# Autodesk Inventor assembly: Controller Asssembly
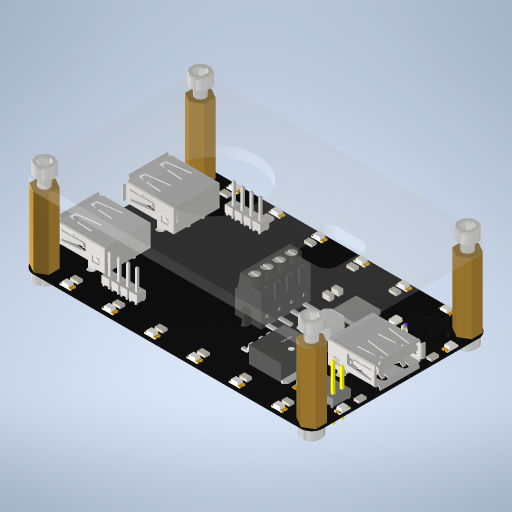
[picture p0: Inventor's stored thumbnail of the model, 512x512]
Saved by Autodesk Inventor 2023 (Build 270158000, 158)
## iProperties
Created: 2022-08-29
Part Number: Controller Asssembly
Document SubType Name: Assembly
Designer: swift
Author: swift
## Documents named in this file (5)
- C:\Users\swift\workspace\fairy-light-controller\Controller Cover\Controller Asssembly.iam
- C:\Users\swift\workspace\fairy-light-controller\Controller Cover\Fairy_Light_Controller_PCB_v1.ipt
- C:\Users\swift\workspace\fairy-light-controller\Controller Cover\Cover.ipt
- C:\Users\swift\workspace\fairy-light-controller\Controller Cover\Standoff.ipt
- C:\Users\swift\workspace\fairy-light-controller\Controller Cover\M3x6.ipt
## Components (14 placed, 4 different names)
1. Fairy_Light_Controller_PCB_v1:1 — Flush:1, Mate:1, Mate:2, Mate:3, Mate:4, Mate:5, Mate:6, Mate:16, Mate:17, Mate:18, Mate:19, Mate:20, Mate:21, Mate:22, Mate:23
2. Cover:1 — Mate:7, Mate:8, Mate:9, Mate:10, Mate:11, Mate:12, Mate:13, Mate:14, Mate:15
3. Standoff:1 — Flush:1, Flush:2, Mate:7
4. Standoff:2 — Mate:1, Mate:2, Flush:2, Angle:1
5. Standoff:3 — Mate:3, Mate:4, Flush:3
6. Standoff:4 — Mate:5, Mate:6, Flush:3
7. M3x6:1 — Mate:8, Mate:9, Flush:4, Angle:2, Flush:5
8. M3x6:2 — Mate:10, Mate:11, Angle:1, Flush:4, Angle:3, Flush:6
9. M3x6:3 — Mate:12, Mate:13, Angle:2, Flush:7
10. M3x6:4 — Mate:14, Mate:15, Angle:3, Flush:8
11. M3x6:5 — Mate:16, Mate:20, Flush:5
12. M3x6:6 — Mate:17, Mate:21, Flush:6
13. M3x6:7 — Mate:18, Mate:22, Flush:7
14. M3x6:8 — Mate:19, Mate:23, Flush:8
## Relationships (34: Mate 23, Flush 8, Angle 3)
- Flush:1: Fairy_Light_Controller_PCB_v1:1 ↔ Standoff:1
- Mate:1: Fairy_Light_Controller_PCB_v1:1 ↔ Standoff:2
- Mate:2: Fairy_Light_Controller_PCB_v1:1 ↔ Standoff:2
- Flush:2: Standoff:1 ↔ Standoff:2
- Mate:3: Fairy_Light_Controller_PCB_v1:1 ↔ Standoff:3
- Mate:4: Fairy_Light_Controller_PCB_v1:1 ↔ Standoff:3
- Mate:5: Fairy_Light_Controller_PCB_v1:1 ↔ Standoff:4
- Mate:6: Fairy_Light_Controller_PCB_v1:1 ↔ Standoff:4
- Flush:3: Standoff:3 ↔ Standoff:4
- Mate:7: Cover:1 ↔ Standoff:1
- Mate:8: Cover:1 ↔ M3x6:1
- Mate:9: Cover:1 ↔ M3x6:1
- Mate:10: Cover:1 ↔ M3x6:2
- Mate:11: Cover:1 ↔ M3x6:2
- Mate:12: Cover:1 ↔ M3x6:3
- Mate:13: Cover:1 ↔ M3x6:3
- Mate:14: Cover:1 ↔ M3x6:4
- Mate:15: Cover:1 ↔ M3x6:4
- Angle:1 (0 deg): Standoff:2 ↔ M3x6:2
- Flush:4: M3x6:1 ↔ M3x6:2
- Angle:2 (0 deg): M3x6:1 ↔ M3x6:3
- Angle:3 (0 deg): M3x6:2 ↔ M3x6:4
- Mate:16: Fairy_Light_Controller_PCB_v1:1 ↔ M3x6:5
- Mate:17: Fairy_Light_Controller_PCB_v1:1 ↔ M3x6:6
- Mate:18: Fairy_Light_Controller_PCB_v1:1 ↔ M3x6:7
- Mate:19: Fairy_Light_Controller_PCB_v1:1 ↔ M3x6:8
- Mate:20: Fairy_Light_Controller_PCB_v1:1 ↔ M3x6:5
- Mate:21: Fairy_Light_Controller_PCB_v1:1 ↔ M3x6:6
- Mate:22: Fairy_Light_Controller_PCB_v1:1 ↔ M3x6:7
- Mate:23: Fairy_Light_Controller_PCB_v1:1 ↔ M3x6:8
- Flush:5: M3x6:1 ↔ M3x6:5
- Flush:6: M3x6:2 ↔ M3x6:6
- Flush:7: M3x6:3 ↔ M3x6:7
- Flush:8: M3x6:4 ↔ M3x6:8
